# Autodesk Inventor assembly: CHA_007_DrivenPulleyAssembly_MIR1
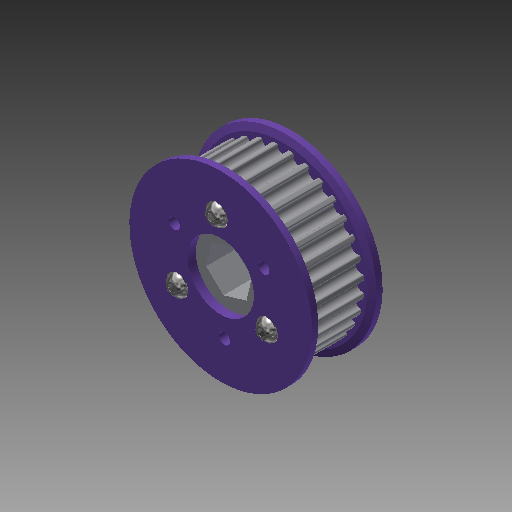
[picture p0: Inventor's stored thumbnail of the model, 512x512]
Saved by Autodesk Inventor 2018 (Build 220112000, 112)
## iProperties
Created: 2020-01-23
Part Number: CHA_007_DrivenPulleyAssembly_MIR1
Document SubType Name: Assembly
Designer: user
Mass: 43.2355 g
Surface Area: 200.66 cm^2
Volume: 37.3013 cm^3
Density: 1.15909 g/cm^3
Author: user
## Documents named in this file (4)
- C:\Users\user\Documents\GrabCAD\New folder\Build season\CHA_007_DrivenPulleyAssembly_MIR1.iam
- C:\Users\user\Documents\GrabCAD\New folder\Build season\CHA_004_DrivePulleyFlange_MIR1.ipt
- C:\Users\user\Documents\GrabCAD\New folder\Build season\CHA_003_DrivePulley_MIR1.ipt
- C:\Users\user\Documents\GrabCAD\New folder\Build season\CHA_008_PulleyScrew(6-32 0.5in)ButtonHeadScrew_MC-91255A148_MIR1.ipt
## Components (9 placed, 3 different names)
1. CHA_004_DrivePulleyFlange_MIR1:1 — Insert:2, Mate:2, Insert:6, Insert:7, Insert:8
2. CHA_003_DrivePulley_MIR1:1 — Insert:2, Mate:2, Mate:1, Insert:1
3. CHA_004_DrivePulleyFlange_MIR1:2 — Mate:1, Insert:1, Insert:3, Insert:4, Insert:5
4. CHA_008_PulleyScrew(6-32 0.5in)ButtonHeadScrew_MC-91255A148_MIR1:1 — Insert:3
5. CHA_008_PulleyScrew(6-32 0.5in)ButtonHeadScrew_MC-91255A148_MIR1:2 — Insert:4
6. CHA_008_PulleyScrew(6-32 0.5in)ButtonHeadScrew_MC-91255A148_MIR1:3 — Insert:5
7. CHA_008_PulleyScrew(6-32 0.5in)ButtonHeadScrew_MC-91255A148_MIR1:4 — Insert:6
8. CHA_008_PulleyScrew(6-32 0.5in)ButtonHeadScrew_MC-91255A148_MIR1:5 — Insert:7
9. CHA_008_PulleyScrew(6-32 0.5in)ButtonHeadScrew_MC-91255A148_MIR1:6 — Insert:8
## Relationships (10: Insert 8, Mate 2)
- Insert:2: CHA_004_DrivePulleyFlange_MIR1:1 ↔ CHA_003_DrivePulley_MIR1:1
- Mate:2: CHA_004_DrivePulleyFlange_MIR1:1 ↔ CHA_003_DrivePulley_MIR1:1
- Mate:1: CHA_003_DrivePulley_MIR1:1 ↔ CHA_004_DrivePulleyFlange_MIR1:2
- Insert:1: CHA_003_DrivePulley_MIR1:1 ↔ CHA_004_DrivePulleyFlange_MIR1:2
- Insert:3: CHA_004_DrivePulleyFlange_MIR1:2 ↔ CHA_008_PulleyScrew(6-32 0.5in)ButtonHeadScrew_MC-91255A148_MIR1:1
- Insert:4: CHA_004_DrivePulleyFlange_MIR1:2 ↔ CHA_008_PulleyScrew(6-32 0.5in)ButtonHeadScrew_MC-91255A148_MIR1:2
- Insert:5: CHA_004_DrivePulleyFlange_MIR1:2 ↔ CHA_008_PulleyScrew(6-32 0.5in)ButtonHeadScrew_MC-91255A148_MIR1:3
- Insert:6: CHA_004_DrivePulleyFlange_MIR1:1 ↔ CHA_008_PulleyScrew(6-32 0.5in)ButtonHeadScrew_MC-91255A148_MIR1:4
- Insert:7: CHA_004_DrivePulleyFlange_MIR1:1 ↔ CHA_008_PulleyScrew(6-32 0.5in)ButtonHeadScrew_MC-91255A148_MIR1:5
- Insert:8: CHA_004_DrivePulleyFlange_MIR1:1 ↔ CHA_008_PulleyScrew(6-32 0.5in)ButtonHeadScrew_MC-91255A148_MIR1:6
